# Autodesk Inventor assembly: zCar
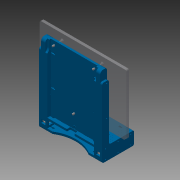
[picture p0: Inventor's stored thumbnail of the model, 180x180]
Saved by Autodesk Inventor 2013 (Build 170138000, 138)
## iProperties
Created: 2015-01-14
Part Number: zCar
Document SubType Name: Assembly
Designer: dzban
Author: dzban
## Documents named in this file (12)
- D:\PIRX\Artisan\OPENSOURCE\ZCar\zCar.iam
- D:\PIRX\Artisan\OPENSOURCE\ZCar\zCarFront.ipt
- D:\PIRX\Artisan\OPENSOURCE\ZCar\zCar_a.ipt
- D:\PIRX\Artisan\OPENSOURCE\StockComponents\LM08UU.ipt
- D:\PIRX\Artisan\OPENSOURCE\ZCar\zCar_b.ipt
- D:\PIRX\Artisan\OPENSOURCE\ZCar\zCar_c.ipt
- D:\PIRX\Artisan\OPENSOURCE\ZCar\zCarNutHolder.ipt
- D:\PIRX\Artisan\OPENSOURCE\ZCar\zCarBack.ipt
- D:\PIRX\Artisan\OPENSOURCE\StockComponents\trapeziodalNut10x2.ipt
- D:\PIRX\Artisan\OPENSOURCE\ZCar\zCarPlate.ipt
- D:\PIRX\Artisan\OPENSOURCE\ZCar\zCarPlexiBed.ipt
- D:\PIRX\Artisan\OPENSOURCE\ZCar\DIN7991x30.ipt
## Components (22 placed, 11 different names)
1. zCarFront:1 — Mate:1, Mate:2, Mate:3, Mate:4, Flush:1, Flush:2, Mate:15, Mate:16, Mate:17, Mate:18, Mate:19, Mate:23
2. zCar_a:1 — Mate:1, Mate:4, Flush:2, Mate:7, Mate:8, Tangent:3, Tangent:4, Tangent:5, Tangent:6, Flush:8, Flush:10, Mate:11, Flush:12, Mate:24
3. zCar_a:2 — Mate:2, Mate:3, Flush:1, Mate:5, Mate:6, Tangent:1, Tangent:2, Tangent:7, Tangent:8, Flush:3, Flush:4, Flush:5, Flush:6, Mate:9, Mate:20, Mate:21, Flush:16, Mate:25
4. LM08UU:1 — Mate:6, Tangent:1, Tangent:8
5. LM08UU:2 — Mate:5, Tangent:2, Tangent:7
6. LM08UU:3 — Mate:8, Tangent:4, Tangent:5
7. LM08UU:4 — Mate:7, Tangent:3, Tangent:6
8. zCar_b:1 — Flush:3, Flush:4, Mate:10, Flush:11, Flush:13, Mate:14
9. zCar_b:2 — Flush:5, Flush:6, Mate:9, Mate:10
10. zCar_b:3 — Flush:7, Flush:9, Mate:12, Flush:14, Mate:13
11. zCar_b:4 — Flush:7, Flush:8, Flush:9, Flush:10, Mate:11, Mate:12
12. zCar_c:1 — Flush:11, Flush:13, Mate:14
13. zCar_c:2 — Flush:12, Flush:14, Mate:13
14. zCarNutHolder:1 — Mate:15, Mate:18, Flush:15, Mate:19
15. zCarNutHolder:2 — Mate:16, Mate:17, Flush:15, Mate:22, Tangent:9, Tangent:10
16. zCarBack:1 — Mate:20, Mate:21, Flush:16
17. trapeziodalNut10x2:1 — Mate:22, Tangent:9, Tangent:10
18. zCarPlate:1 — Mate:23, Mate:24, Mate:25, Insert:1, Insert:2
19. zCarPlexiBed:1 — Insert:1, Insert:2, Insert:3, Insert:4, Insert:5
20. DIN7991x30:1 — Insert:3
21. DIN7991x30:2 — Insert:4
22. DIN7991x30:3 — Insert:5
## Relationships (56: Mate 25, Flush 16, Tangent 10, Insert 5)
- Mate:1: zCarFront:1 ↔ zCar_a:1
- Mate:2: zCarFront:1 ↔ zCar_a:2
- Mate:3: zCarFront:1 ↔ zCar_a:2
- Mate:4: zCarFront:1 ↔ zCar_a:1
- Flush:1: zCarFront:1 ↔ zCar_a:2
- Flush:2: zCarFront:1 ↔ zCar_a:1
- Mate:5: zCar_a:2 ↔ LM08UU:2
- Mate:6: zCar_a:2 ↔ LM08UU:1
- Tangent:1: zCar_a:2 ↔ LM08UU:1
- Tangent:2: zCar_a:2 ↔ LM08UU:2
- Mate:7: zCar_a:1 ↔ LM08UU:4
- Mate:8: zCar_a:1 ↔ LM08UU:3
- Tangent:3: zCar_a:1 ↔ LM08UU:4
- Tangent:4: zCar_a:1 ↔ LM08UU:3
- Tangent:5: zCar_a:1 ↔ LM08UU:3
- Tangent:6: zCar_a:1 ↔ LM08UU:4
- Tangent:7: zCar_a:2 ↔ LM08UU:2
- Tangent:8: zCar_a:2 ↔ LM08UU:1
- Flush:3: zCar_a:2 ↔ zCar_b:1
- Flush:4: zCar_a:2 ↔ zCar_b:1
- Flush:5: zCar_a:2 ↔ zCar_b:2
- Flush:6: zCar_a:2 ↔ zCar_b:2
- Mate:9: zCar_a:2 ↔ zCar_b:2
- Mate:10: zCar_b:1 ↔ zCar_b:2
- Flush:7: zCar_b:3 ↔ zCar_b:4
- Flush:8: zCar_a:1 ↔ zCar_b:4
- Flush:9: zCar_b:3 ↔ zCar_b:4
- Flush:10: zCar_a:1 ↔ zCar_b:4
- Mate:11: zCar_a:1 ↔ zCar_b:4
- Mate:12: zCar_b:3 ↔ zCar_b:4
- Flush:11: zCar_b:1 ↔ zCar_c:1
- Flush:12: zCar_a:1 ↔ zCar_c:2
- Flush:13: zCar_b:1 ↔ zCar_c:1
- Flush:14: zCar_b:3 ↔ zCar_c:2
- Mate:13: zCar_b:3 ↔ zCar_c:2
- Mate:14: zCar_b:1 ↔ zCar_c:1
- Mate:15: zCarFront:1 ↔ zCarNutHolder:1
- Mate:16: zCarFront:1 ↔ zCarNutHolder:2
- Mate:17: zCarFront:1 ↔ zCarNutHolder:2
- Mate:18: zCarFront:1 ↔ zCarNutHolder:1
- Flush:15: zCarNutHolder:1 ↔ zCarNutHolder:2
- Mate:19: zCarFront:1 ↔ zCarNutHolder:1
- Mate:20: zCar_a:2 ↔ zCarBack:1
- Mate:21: zCar_a:2 ↔ zCarBack:1
- Flush:16: zCar_a:2 ↔ zCarBack:1
- Mate:22: zCarNutHolder:2 ↔ trapeziodalNut10x2:1
- Tangent:9: zCarNutHolder:2 ↔ trapeziodalNut10x2:1
- Tangent:10: zCarNutHolder:2 ↔ trapeziodalNut10x2:1
- Mate:23: zCarFront:1 ↔ zCarPlate:1
- Mate:24: zCar_a:1 ↔ zCarPlate:1
- Mate:25: zCar_a:2 ↔ zCarPlate:1
- Insert:1 (10 mm): zCarPlate:1 ↔ zCarPlexiBed:1
- Insert:2 (10 mm): zCarPlate:1 ↔ zCarPlexiBed:1
- Insert:3: zCarPlexiBed:1 ↔ DIN7991x30:1
- Insert:4: zCarPlexiBed:1 ↔ DIN7991x30:2
- Insert:5: zCarPlexiBed:1 ↔ DIN7991x30:3
